# Autodesk Inventor assembly: BearingHousing
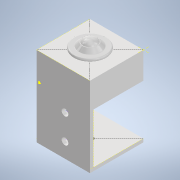
[picture p0: Inventor's stored thumbnail of the model, 180x180]
Saved by Autodesk Inventor 2020 (Build 240168000, 168)
## iProperties
Created: 2021-12-14
Part Number: BearingHousing
Document SubType Name: Assembly
Designer: danie
Author: danie
## Documents named in this file (3)
- C:\Users\danie\Documents\Capstone\Solidworks\BearingHousing.iam
- C:\Users\danie\Downloads\6421K66_Press-Fit Ball Transfer.ipt
- C:\Users\danie\Documents\Capstone\Solidworks\Bearing Housing.ipt
## Components (2 placed, 2 different names)
1. 6421K66_Press-Fit Ball Transfer:1 — Slider:1
2. Bearing Housing:1 — Slider:1
## Relationships (1: TranslationJoint 1)
- Slider:1 [TranslationJoint] (-8.89 mm): 6421K66_Press-Fit Ball Transfer:1 ↔ Bearing Housing:1
